# Autodesk Inventor assembly: COP315_Lock
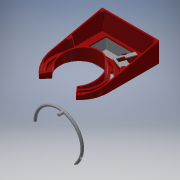
[picture p0: Inventor's stored thumbnail of the model, 180x180]
Saved by Autodesk Inventor 2018 (Build 220112000, 112)
## iProperties
Created: 2018-04-13
Part Number: COP315_Lock
Document SubType Name: Assembly
Designer: anshs
Author: anshs
## Documents named in this file (7)
- F:\COP315\COP315_Lock.iam
- F:\COP315\cop315_part1_2_upper.ipt
- F:\COP315\cop315_part1_2.ipt
- F:\COP315\Motor_cover.ipt
- F:\COP315\Cover_strip_left.ipt
- F:\COP315\Extrusion.ipt
- C:\Users\anshs\Desktop\Ring.ipt
## Components (7 placed, 6 different names)
1. cop315_part1_2_upper:1 — Mate:7, Insert:5, Insert:6
2. cop315_part1_2:1 — Mate:5, Insert:1, Insert:2, Mate:6, Insert:3, Insert:4, Mate:7, Insert:5, Insert:6, Mate:8, Mate:9, Mate:10, Mate:11, Mate:12, Flush:3
3. Motor_cover:1 — Mate:11, Mate:12, Flush:3
4. Cover_strip_left:1 — Mate:5, Insert:1, Insert:2
5. Cover_strip_left:2 — Mate:6, Insert:3, Insert:4
6. Extrusion:1 — Mate:8, Mate:9, Mate:10
7. Ring:1
## Relationships (15: Mate 8, Insert 6, Flush 1)
- Mate:5: cop315_part1_2:1 ↔ Cover_strip_left:1
- Insert:1: cop315_part1_2:1 ↔ Cover_strip_left:1
- Insert:2: cop315_part1_2:1 ↔ Cover_strip_left:1
- Mate:6: cop315_part1_2:1 ↔ Cover_strip_left:2
- Insert:3: cop315_part1_2:1 ↔ Cover_strip_left:2
- Insert:4: cop315_part1_2:1 ↔ Cover_strip_left:2
- Mate:7: cop315_part1_2_upper:1 ↔ cop315_part1_2:1
- Insert:5: cop315_part1_2_upper:1 ↔ cop315_part1_2:1
- Insert:6: cop315_part1_2_upper:1 ↔ cop315_part1_2:1
- Mate:8: cop315_part1_2:1 ↔ Extrusion:1
- Mate:9: cop315_part1_2:1 ↔ Extrusion:1
- Mate:10: cop315_part1_2:1 ↔ Extrusion:1
- Mate:11: cop315_part1_2:1 ↔ Motor_cover:1
- Mate:12: cop315_part1_2:1 ↔ Motor_cover:1
- Flush:3 (2 mm): cop315_part1_2:1 ↔ Motor_cover:1
